# Autodesk Inventor assembly: croixCatcher
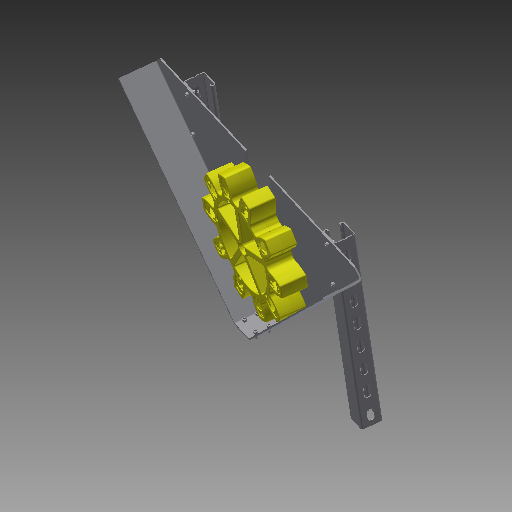
[picture p0: Inventor's stored thumbnail of the model, 512x512]
Saved by Autodesk Inventor 2017 (Build 210142000, 142)
## iProperties
Created: 2017-01-21
Part Number: croixCatcher
Document SubType Name: Assembly
Designer: kingb
Author: kingb
## Documents named in this file (5)
- C:\Users\kingb\Desktop\CAD\croixCatcher.iam
- C:\Users\kingb\Desktop\CAD\scoreGear.iam
- C:\Users\kingb\Desktop\CAD\gearCatch.ipt
- C:\Users\kingb\Desktop\CAD\10-32x0500_shcs_HX-SHCS 0.19-32x1.375x1-C.ipt
- C:\Users\kingb\Desktop\CAD\3230T450_STRUT CHANNEL.ipt
## Components (12 placed, 4 different names)
1. scoreGear:1 [sub-assembly]
2. gearCatch:1
3. 10-32x0500_shcs_HX-SHCS 0.19-32x1.375x1-C:1
4. 10-32x0500_shcs_HX-SHCS 0.19-32x1.375x1-C:2
5. 10-32x0500_shcs_HX-SHCS 0.19-32x1.375x1-C:3
6. 10-32x0500_shcs_HX-SHCS 0.19-32x1.375x1-C:4
7. 3230T450_STRUT CHANNEL:1
8. 3230T450_STRUT CHANNEL:2
9. 10-32x0500_shcs_HX-SHCS 0.19-32x1.375x1-C:5
10. 10-32x0500_shcs_HX-SHCS 0.19-32x1.375x1-C:6
11. 10-32x0500_shcs_HX-SHCS 0.19-32x1.375x1-C:7
12. 10-32x0500_shcs_HX-SHCS 0.19-32x1.375x1-C:8
## Relationships (5: Tangent 3, Mate 2)
- [Tangent]: scoreGear:1 ↔ gearCatch:1
- [Tangent]: scoreGear:1 ↔ gearCatch:1
- [Tangent]: scoreGear:1 ↔ gearCatch:1
- [Mate]: gearCatch:1 ↔ 3230T450_STRUT CHANNEL:2
- [Mate]: gearCatch:1 ↔ 3230T450_STRUT CHANNEL:1
